# Autodesk Inventor assembly: Frame
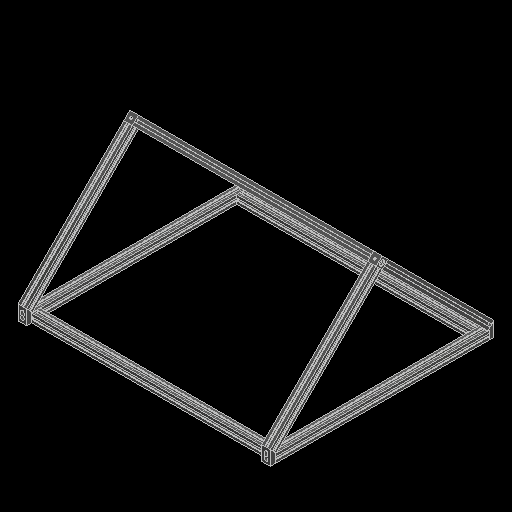
[picture p0: Inventor's stored thumbnail of the model, 512x512]
Saved by Autodesk Inventor 2023 (Build 270158000, 158)
## iProperties
Created: 2023-07-18
Part Number: Frame
Document SubType Name: Assembly
Designer: tandu
Author: tandu
Revision Number: ANY
## Documents named in this file (6)
- C:\Users\tandu\Documents\GrabCAD\Custom Conveyor Belt 3D Printer\V1\Parts\Frame\printer_largeeeFrame.iam
- C:\Users\tandu\Documents\GrabCAD\Custom Conveyor Belt 3D Printer\V1\Parts\Frame\printer_largeee500mm_extrusion.ipt
- C:\Users\tandu\Documents\GrabCAD\Custom Conveyor Belt 3D Printer\V1\Parts\Frame\printer_largeee350mm_extrusion.ipt
- C:\Users\tandu\Documents\GrabCAD\Custom Conveyor Belt 3D Printer\V1\Parts\Frame\printer_largeeecube.ipt
- C:\Users\tandu\Documents\GrabCAD\Custom Conveyor Belt 3D Printer\V1\Parts\Frame\printer_largeeeangle_corner_connector_large.ipt
- C:\Users\tandu\Documents\GrabCAD\Custom Conveyor Belt 3D Printer\V1\Parts\Frame\Width Extrusion.ipt
## Components (15 placed, 11 different names)
1. width extrusion:5 — Insert:11, Flush:11, Insert:12, Flush:12
2. width extrusion:6 — Mate:2, Flush:16, Flush:17
3. width extrusion:7 — Flush:14, Flush:15, Mate:3
4. 500mm_extrusion_333 — Insert:1, Flush:1, Insert:4, Flush:4, Flush:15, Mate:2, Flush:16, Flush:17, Mate:3
5. 350mm_extrusion_336 — Insert:5, Flush:5
6. 350mm_extrusion_337 — Insert:2, Flush:2, Insert:3, Flush:3
7. cube_339 — Insert:3, Flush:3, Insert:11, Flush:11
8. angle_corner_connector_large_344 — Insert:1, Flush:1, Insert:2, Flush:2
9. angle_corner_connector_large_346 — Insert:4, Flush:4, Insert:5, Flush:5, Flush:14
10. printer_largeee500mm_extrusion:2
11. 350 mm extrusion:8
12. 350 mm extrusion:9
13. printer_largeeecube:2 — Insert:12, Flush:12
14. printer_largeeeangle_corner_connector_large:4
15. printer_largeeeangle_corner_connector_large:5
## Relationships (30: Flush 16, Insert 12, Mate 2)
- Insert:1: 500mm_extrusion_333 ↔ angle_corner_connector_large_344
- Flush:1: 500mm_extrusion_333 ↔ angle_corner_connector_large_344
- Insert:2: 350mm_extrusion_337 ↔ angle_corner_connector_large_344
- Flush:2: 350mm_extrusion_337 ↔ angle_corner_connector_large_344
- Insert:3: 350mm_extrusion_337 ↔ cube_339
- Flush:3: 350mm_extrusion_337 ↔ cube_339
- Insert:4: 500mm_extrusion_333 ↔ angle_corner_connector_large_346
- Flush:4: 500mm_extrusion_333 ↔ angle_corner_connector_large_346
- Insert:5: 350mm_extrusion_336 ↔ angle_corner_connector_large_346
- Flush:5: 350mm_extrusion_336 ↔ angle_corner_connector_large_346
- [Insert]: printer_largeee500mm_extrusion:2 ↔ printer_largeeeangle_corner_connector_large:4
- [Flush]: printer_largeee500mm_extrusion:2 ↔ printer_largeeeangle_corner_connector_large:4
- [Insert]: 350 mm extrusion:9 ↔ printer_largeeeangle_corner_connector_large:4
- [Flush]: 350 mm extrusion:9 ↔ printer_largeeeangle_corner_connector_large:4
- [Insert]: 350 mm extrusion:9 ↔ printer_largeeecube:2
- [Flush]: 350 mm extrusion:9 ↔ printer_largeeecube:2
- [Insert]: printer_largeee500mm_extrusion:2 ↔ printer_largeeeangle_corner_connector_large:5
- [Flush]: printer_largeee500mm_extrusion:2 ↔ printer_largeeeangle_corner_connector_large:5
- [Insert]: 350 mm extrusion:8 ↔ printer_largeeeangle_corner_connector_large:5
- [Flush]: 350 mm extrusion:8 ↔ printer_largeeeangle_corner_connector_large:5
- Insert:11: width extrusion:5 ↔ cube_339
- Flush:11: width extrusion:5 ↔ cube_339
- Insert:12: width extrusion:5 ↔ printer_largeeecube:2
- Flush:12: width extrusion:5 ↔ printer_largeeecube:2
- Flush:14: width extrusion:7 ↔ angle_corner_connector_large_346
- Flush:15: width extrusion:7 ↔ 500mm_extrusion_333
- Mate:2: width extrusion:6 ↔ 500mm_extrusion_333
- Flush:16: width extrusion:6 ↔ 500mm_extrusion_333
- Flush:17: width extrusion:6 ↔ 500mm_extrusion_333
- Mate:3: width extrusion:7 ↔ 500mm_extrusion_333
## Named parameters: d10_d0 = 0 mm, d11_d1 = 0 mm, d12_d2 = 0 mm, d13_d3 = 0 mm, d14_d4 = 0 mm, d15_d5 = 0 mm, d16_d6 = 0 mm, d17_d7 = 0 mm, d18_d8 = 0 mm, d19_d9 = 0 mm
